# Autodesk Inventor assembly: Driver Board Mount HSI
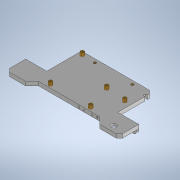
[picture p0: Inventor's stored thumbnail of the model, 180x180]
Saved by Autodesk Inventor 2022 (Build 260153000, 153)
## iProperties
Created: 2022-06-07
Part Number: Driver Board Mount HSI
Document SubType Name: Assembly
Designer: Nick
Author: Nick
## Documents named in this file (4)
- Y:\Projects\Mini_Sand_Table\Driver Board Mount HSI.iam
- Y:\Projects\Mini_Sand_Table\Motor Side Foot.ipt
- Y:\Projects\Mini_Sand_Table\M3 Heat Set Inserts.ipt
- Y:\Projects\Mini_Sand_Table\5mm M3 Brass Standoff.ipt
## Components (13 placed, 3 different names)
1. Motor Side Foot:1 — Insert:1, Insert:2, Insert:3, Insert:4, Insert:5, Insert:6, Insert:7
2. M3 Heat Set Inserts:1 — Insert:1, Insert:8
3. M3 Heat Set Inserts:2 — Insert:3, Insert:10
4. M3 Heat Set Inserts:3 — Insert:2, Insert:9
5. M3 Heat Set Inserts:4 — Insert:4, Insert:11
6. M3 Heat Set Inserts:5 — Insert:5, Insert:12
7. M3 Heat Set Inserts:6 — Insert:6
8. M3 Heat Set Inserts:7 — Insert:7
9. 5mm M3 Brass Standoff:1 — Insert:9
10. 5mm M3 Brass Standoff:2 — Insert:11
11. 5mm M3 Brass Standoff:3 — Insert:8
12. 5mm M3 Brass Standoff:4 — Insert:12
13. 5mm M3 Brass Standoff:5 — Insert:10
## Relationships (12: Insert 12)
- Insert:1: Motor Side Foot:1 ↔ M3 Heat Set Inserts:1
- Insert:2: Motor Side Foot:1 ↔ M3 Heat Set Inserts:3
- Insert:3: Motor Side Foot:1 ↔ M3 Heat Set Inserts:2
- Insert:4: Motor Side Foot:1 ↔ M3 Heat Set Inserts:4
- Insert:5: Motor Side Foot:1 ↔ M3 Heat Set Inserts:5
- Insert:6: Motor Side Foot:1 ↔ M3 Heat Set Inserts:6
- Insert:7: Motor Side Foot:1 ↔ M3 Heat Set Inserts:7
- Insert:8: M3 Heat Set Inserts:1 ↔ 5mm M3 Brass Standoff:3
- Insert:9: M3 Heat Set Inserts:3 ↔ 5mm M3 Brass Standoff:1
- Insert:10: M3 Heat Set Inserts:2 ↔ 5mm M3 Brass Standoff:5
- Insert:11: M3 Heat Set Inserts:4 ↔ 5mm M3 Brass Standoff:2
- Insert:12: M3 Heat Set Inserts:5 ↔ 5mm M3 Brass Standoff:4
